# Autodesk Inventor assembly: Assembly_Matchboxscope_injectionmolded_ESPectrometer
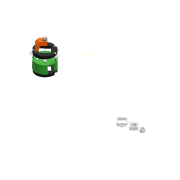
[picture p0: Inventor's stored thumbnail of the model, 180x180]
Saved by Autodesk Inventor 2022 (Build 260153000, 153)
## iProperties
Created: 2023-04-12
Part Number: Assembly_Matchboxscope_injectionmolded_ESPectrometer
Document SubType Name: Assembly
Designer: diederichbenedict
Author: diederichbenedict
## Documents named in this file (14)
- C:\Users\diederichbenedict\Dropbox\Dokumente\Promotion\PROJECTS\Matchboxscope\INVENTOR\RELEASE\InjectionMolded\Assembly_Matchboxscope_injectionmolded_ESPectrometer.iam
- C:\Users\diederichbenedict\Dropbox\Dokumente\Promotion\PROJECTS\Matchboxscope\INVENTOR\RELEASE\InjectionMolded\IM_Matchboxscope_base.ipt
- C:\Users\diederichbenedict\Dropbox\Dokumente\Promotion\PROJECTS\Matchboxscope\INVENTOR\RELEASE\InjectionMolded\IM_Matchboxscope_plate.ipt
- C:\Users\diederichbenedict\Dropbox\Dokumente\Promotion\PROJECTS\Matchboxscope\INVENTOR\RELEASE\InjectionMolded\IM_Lensholder.ipt
- C:\Users\diederichbenedict\Dropbox\Dokumente\Promotion\PROJECTS\Matchboxscope\INVENTOR\RELEASE\InjectionMolded\IM_Periscope.ipt
- C:\Users\diederichbenedict\Dropbox\Dokumente\Promotion\PROJECTS\Matchboxscope\INVENTOR\RELEASE\InjectionMolded\IM_ledholder.ipt
- C:\Users\diederichbenedict\Dropbox\Dokumente\Promotion\PROJECTS\Matchboxscope\INVENTOR\RELEASE\InjectionMolded\Anglerfish_Cameraspacer.ipt
- C:\Users\diederichbenedict\Dropbox\Dokumente\Promotion\PROJECTS\Matchboxscope\INVENTOR\RELEASE\InjectionMolded\00_CCTV_M12_VCM_large.ipt
- C:\Users\diederichbenedict\Dropbox\Dokumente\Promotion\PROJECTS\Matchboxscope\INVENTOR\RELEASE\InjectionMolded\IM_Lensholder_M12.ipt
- C:\Users\diederichbenedict\Dropbox\Dokumente\Promotion\PROJECTS\Matchboxscope\INVENTOR\RELEASE\InjectionMolded\Matchboxscope_M12_Lensadapter_v0.ipt
- C:\Users\diederichbenedict\Dropbox\Dokumente\Promotion\PROJECTS\Matchboxscope\INVENTOR\RELEASE\InjectionMolded\00_Turningscrew.ipt
- C:\Users\diederichbenedict\Documents\Inventor\Content Center Files\R2022\de-DE\DIN 912\DIN 912 - M3 x 0.5 x 25 x 18.ipt
- C:\Users\diederichbenedict\Documents\Inventor\Content Center Files\R2022\de-DE\DIN 912\DIN 912 - M3 x 0.5 x 10 x 8.75.ipt
- C:\Users\diederichbenedict\Dropbox\Dokumente\Promotion\PROJECTS\Matchboxscope\INVENTOR\RELEASE\InjectionMolded\00_LED_lamp.ipt
## Components (20 placed, 13 different names)
1. IM_Matchboxscope_base:1 — Fluchtend:1, Einfügen:3, Passend:3
2. IM_Matchboxscope_plate:1 — Einfügen:10
3. IM_Lensholder:1 — Fluchtend:1, Einfügen:8
4. IM_Periscope:1
5. IM_ledholder:1 — Einfügen:4, Einfügen:9, Einfügen:14
6. Anglerfish_Cameraspacer:1
7. 00_CCTV_M12_VCM_large:1 — Passend:2, Winkel:2
8. IM_Lensholder_M12:1 — Passend:2, Winkel:2
9. Matchboxscope_M12_Lensadapter_v0:1
10. 00_Turningscrew:1 — Einfügen:11
11. IM_Matchboxscope_plate:2 — Einfügen:3, Passend:3, Einfügen:4, Einfügen:5, Einfügen:6, Einfügen:7, Einfügen:11, Einfügen:12, Einfügen:13
12. DIN 912 - ersetzt durch DIN EN ISO 4762 M3 x 25:1 — Einfügen:5
13. DIN 912 - ersetzt durch DIN EN ISO 4762 M3 x 25:2 — Einfügen:6
14. DIN 912 - ersetzt durch DIN EN ISO 4762 M3 x 25:3 — Einfügen:7
15. DIN 912 - ersetzt durch DIN EN ISO 4762 M3 x 10:1 — Einfügen:10
16. DIN 912 - ersetzt durch DIN EN ISO 4762 M3 x 10:2 — Einfügen:9
17. DIN 912 - ersetzt durch DIN EN ISO 4762 M3 x 10:3 — Einfügen:8
18. 00_Turningscrew:2 — Einfügen:13
19. 00_Turningscrew:3 — Einfügen:12
20. 00_LED_lamp:1 — Einfügen:14
## Relationships (18: Insert 14, Mate 2, Flush 1, Angle 1)
- [Insert]: IM_Matchboxscope_base:1 ↔ IM_Matchboxscope_plate:1
- [Insert]: IM_Matchboxscope_base:1 ↔ IM_Matchboxscope_plate:1
- Fluchtend:1 [Flush]: IM_Matchboxscope_base:1 ↔ IM_Lensholder:1
- Passend:2 [Mate]: 00_CCTV_M12_VCM_large:1 ↔ IM_Lensholder_M12:1
- Winkel:2 [Angle] (45 deg): 00_CCTV_M12_VCM_large:1 ↔ IM_Lensholder_M12:1
- Einfügen:3 [Insert] (15 mm): IM_Matchboxscope_base:1 ↔ IM_Matchboxscope_plate:2
- Passend:3 [Mate]: IM_Matchboxscope_base:1 ↔ IM_Matchboxscope_plate:2
- Einfügen:4 [Insert]: IM_ledholder:1 ↔ IM_Matchboxscope_plate:2
- Einfügen:5 [Insert]: IM_Matchboxscope_plate:2 ↔ DIN 912 - ersetzt durch DIN EN ISO 4762 M3 x 25:1
- Einfügen:6 [Insert]: IM_Matchboxscope_plate:2 ↔ DIN 912 - ersetzt durch DIN EN ISO 4762 M3 x 25:2
- Einfügen:7 [Insert]: IM_Matchboxscope_plate:2 ↔ DIN 912 - ersetzt durch DIN EN ISO 4762 M3 x 25:3
- Einfügen:8 [Insert]: IM_Lensholder:1 ↔ DIN 912 - ersetzt durch DIN EN ISO 4762 M3 x 10:3
- Einfügen:9 [Insert]: IM_ledholder:1 ↔ DIN 912 - ersetzt durch DIN EN ISO 4762 M3 x 10:2
- Einfügen:10 [Insert] (-4 mm): IM_Matchboxscope_plate:1 ↔ DIN 912 - ersetzt durch DIN EN ISO 4762 M3 x 10:1
- Einfügen:11 [Insert]: 00_Turningscrew:1 ↔ IM_Matchboxscope_plate:2
- Einfügen:12 [Insert]: IM_Matchboxscope_plate:2 ↔ 00_Turningscrew:3
- Einfügen:13 [Insert]: IM_Matchboxscope_plate:2 ↔ 00_Turningscrew:2
- Einfügen:14 [Insert]: IM_ledholder:1 ↔ 00_LED_lamp:1
